# Autodesk Inventor assembly: Shifter v2
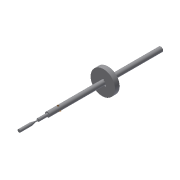
[picture p0: Inventor's stored thumbnail of the model, 180x180]
Saved by Autodesk Inventor 2014 (Build 180170000, 170)
## iProperties
Created: 2014-02-23
Part Number: Shifter v2
Document SubType Name: Assembly
Designer: Owner
Author: Owner
## Documents named in this file (5)
- C:\Users\Owner\Documents\Inventor\FRC 2014\Frc Chassis 2014\Shifter v2.iam
- C:\Users\Owner\Documents\Inventor\FRC 2014\Frc Chassis 2014\transmission plunger.ipt
- C:\Users\Owner\Documents\Inventor\FRC 2014\Frc Chassis 2014\augmented gear v3.ipt
- C:\Users\Owner\Documents\Inventor\FRC 2014\Frc Chassis 2014\Ball bearing - .1875.ipt
- C:\Users\Owner\Documents\Inventor\FRC 2014\Frc Chassis 2014\transmission tube v1.ipt
## Components (6 placed, 4 different names)
1. transmission plunger:1 — Insert:1
2. augmented gear v3:1 — Tangent:1, Tangent:2, Tangent:3
3. Ball bearing - .1875:1 — Tangent:5
4. Ball bearing - .1875:2 — Tangent:6
5. Ball bearing - .1875:3 — Tangent:4
6. transmission tube v1:1 — Insert:1, Tangent:1, Tangent:2, Tangent:3, Tangent:4, Tangent:5, Tangent:6
## Relationships (7: Tangent 6, Insert 1)
- Insert:1: transmission plunger:1 ↔ transmission tube v1:1
- Tangent:1: augmented gear v3:1 ↔ transmission tube v1:1
- Tangent:2: augmented gear v3:1 ↔ transmission tube v1:1
- Tangent:3: augmented gear v3:1 ↔ transmission tube v1:1
- Tangent:4: Ball bearing - .1875:3 ↔ transmission tube v1:1
- Tangent:5: Ball bearing - .1875:1 ↔ transmission tube v1:1
- Tangent:6: Ball bearing - .1875:2 ↔ transmission tube v1:1
